# Autodesk Inventor assembly: base_herramienta
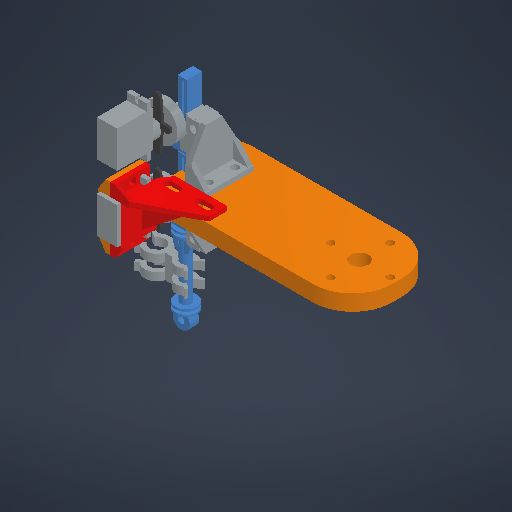
[picture p0: Inventor's stored thumbnail of the model, 512x512]
Saved by Autodesk Inventor 2026.2 (Build 302298000, 298)
## iProperties
Created: 2024-10-01
Part Number: base_herramienta
Document SubType Name: Assembly
Designer: User
Author: User
## Documents named in this file (5)
- E:\Proyectos\scara-robot-rrp\mechanical\inventor\base_herramienta.iam
- E:\Proyectos\scara-robot-rrp\mechanical\inventor\pinza.iam
- E:\Proyectos\scara-robot-rrp\mechanical\inventor\soporte-motor.ipt
- E:\Proyectos\scara-robot-rrp\mechanical\inventor\soprte_motor.ipt
- E:\Proyectos\scara-robot-rrp\mechanical\inventor\lamina_herrAMIENTA.ipt
## Components (4 placed, 4 different names)
1. pinza:1 [sub-assembly] — Mate:2, Mate:3, Flush:3, Mate:4, Mate:5, Mate:6
2. soporte-motor:1 — Mate:1, Flush:1, Flush:2, Mate:3, Flush:3
3. soprte_motor:1 — Mate:1, Flush:1, Flush:2, Mate:2
4. lamina_herrAMIENTA:1 — Mate:4, Mate:5, Mate:6
## Relationships (9: Mate 6, Flush 3)
- Mate:1: soporte-motor:1 ↔ soprte_motor:1
- Flush:1: soporte-motor:1 ↔ soprte_motor:1
- Flush:2: soporte-motor:1 ↔ soprte_motor:1
- Mate:2: pinza:1 ↔ soprte_motor:1
- Mate:3: pinza:1 ↔ soporte-motor:1
- Flush:3 (2.34 mm): pinza:1 ↔ soporte-motor:1
- Mate:4 (-8 mm): pinza:1 ↔ lamina_herrAMIENTA:1
- Mate:5: pinza:1 ↔ lamina_herrAMIENTA:1
- Mate:6: pinza:1 ↔ lamina_herrAMIENTA:1
